# Autodesk Inventor assembly: Overview
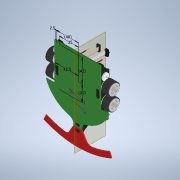
[picture p0: Inventor's stored thumbnail of the model, 180x180]
Saved by Autodesk Inventor 2022 (Build 260153000, 153)
## iProperties
Created: 2021-10-05
Part Number: Overview
Document SubType Name: Assembly
Designer: shiok
Mass: 103.359 g
Surface Area: 978.929 cm^2
Volume: 78.8399 cm^3
Density: 1.311 g/cm^3
Author: shiok
## Documents named in this file (11)
- C:\Users\Yazawa\Documents\GitHub\murakumo\inventor\Overview.iam
- C:\Users\Yazawa\Documents\GitHub\murakumo\inventor\flame.ipt
- C:\Users\Yazawa\Documents\GitHub\murakumo\inventor\Motor.iam
- C:\Users\Yazawa\Documents\GitHub\murakumo\inventor\Motor_MIR1.iam
- C:\Users\Yazawa\Documents\GitHub\murakumo\inventor\top.ipt
- C:\Users\Yazawa\Documents\GitHub\murakumo\inventor\sensorbar.ipt
- C:\Users\Yazawa\Documents\GitHub\murakumo\inventor\sensor.ipt
- C:\Users\Yazawa\Documents\GitHub\murakumo\inventor\SideSensor.ipt
- C:\Users\Yazawa\Documents\GitHub\murakumo\inventor\SideSensorCircuit.ipt
- C:\Users\Yazawa\Documents\GitHub\murakumo\inventor\SideSensor_MIR.ipt
- C:\Users\Yazawa\Documents\GitHub\murakumo\inventor\SideSensorCircuit_MIR1.ipt
## Components (10 placed, 10 different names)
1. flame:1 — フラッシュ:1, フラッシュ:2, フラッシュ:3, 挿入:2, メイト:2, 挿入:17
2. Motor:1 [sub-assembly] — 挿入:2, メイト:2, 挿入:3, メイト:3, 挿入:13
3. top:1 — メイト:1, 挿入:3, 挿入:4, メイト:3, メイト:4, 挿入:5, 挿入:6
4. sensorbar:1 — フラッシュ:7, メイト:4, 挿入:5, 挿入:6, 挿入:7, 挿入:8, メイト:5
5. sensor:1 — フラッシュ:6, 挿入:7, 挿入:8, メイト:5
6. Motor_MIR1:1 [sub-assembly] — 挿入:4, 挿入:14, メイト:8, 挿入:17
7. SideSensor:1 — 挿入:11, 挿入:12, メイト:7, 挿入:13
8. SideSensorCircuit:1 — 挿入:11, 挿入:12, メイト:7
9. SideSensor_MIR:1 — 挿入:14, メイト:8, 挿入:15, 挿入:16, メイト:9
10. SideSensorCircuit_MIR1:1 — 挿入:15, 挿入:16, メイト:9
## Relationships (27: Insert 14, Mate 8, Flush 5)
- フラッシュ:1 [Flush]: flame:1
- フラッシュ:2 [Flush]: flame:1
- フラッシュ:3 [Flush]: flame:1
- メイト:1 [Mate]: top:1
- フラッシュ:6 [Flush]: sensor:1
- フラッシュ:7 [Flush]: sensorbar:1
- 挿入:2 [Insert]: flame:1 ↔ Motor:1
- メイト:2 [Mate]: flame:1 ↔ Motor:1
- 挿入:3 [Insert]: Motor:1 ↔ top:1
- 挿入:4 [Insert]: top:1 ↔ Motor_MIR1:1
- メイト:3 [Mate]: Motor:1 ↔ top:1
- メイト:4 [Mate]: top:1 ↔ sensorbar:1
- 挿入:5 [Insert]: top:1 ↔ sensorbar:1
- 挿入:6 [Insert]: top:1 ↔ sensorbar:1
- 挿入:7 [Insert]: sensorbar:1 ↔ sensor:1
- 挿入:8 [Insert]: sensorbar:1 ↔ sensor:1
- メイト:5 [Mate]: sensorbar:1 ↔ sensor:1
- 挿入:11 [Insert]: SideSensor:1 ↔ SideSensorCircuit:1
- 挿入:12 [Insert]: SideSensor:1 ↔ SideSensorCircuit:1
- メイト:7 [Mate]: SideSensor:1 ↔ SideSensorCircuit:1
- 挿入:13 [Insert]: Motor:1 ↔ SideSensor:1
- 挿入:14 [Insert]: Motor_MIR1:1 ↔ SideSensor_MIR:1
- メイト:8 [Mate]: Motor_MIR1:1 ↔ SideSensor_MIR:1
- 挿入:15 [Insert]: SideSensor_MIR:1 ↔ SideSensorCircuit_MIR1:1
- 挿入:16 [Insert]: SideSensor_MIR:1 ↔ SideSensorCircuit_MIR1:1
- メイト:9 [Mate]: SideSensor_MIR:1 ↔ SideSensorCircuit_MIR1:1
- 挿入:17 [Insert]: flame:1 ↔ Motor_MIR1:1
